# Autodesk Inventor assembly: CapStone Assembly
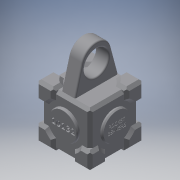
[picture p0: Inventor's stored thumbnail of the model, 180x180]
Saved by Autodesk Inventor 2018 (Build 220112000, 112)
## iProperties
Created: 2020-01-10
Part Number: CapStone Assembly
Document SubType Name: Assembly
Designer: AOFUser
Author: AOFUser
## Documents named in this file (3)
- C:\Users\AOFUser\Documents\GitHub\3D-Models\Robotics\CapStone\CapStone Assembly.iam
- C:\Users\AOFUser\Documents\GitHub\3D-Models\Robotics\CapStone\CapStone.ipt
- C:\Users\AOFUser\Documents\GitHub\3D-Models\Robotics\CapStone\CapStone Handle.ipt
## Components (2 placed, 2 different names)
1. CapStone:1 — Rigid:1
2. CapStone Handle:1 — Rigid:1
## Relationships (1: WeldJoint 1)
- Rigid:1 [WeldJoint]: CapStone:1 ↔ CapStone Handle:1
